# Autodesk Inventor assembly: promo
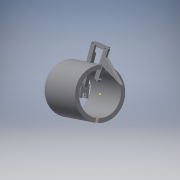
[picture p0: Inventor's stored thumbnail of the model, 180x180]
Saved by Autodesk Inventor 2016 (Build 200138000, 138)
## iProperties
Created: 2016-05-12
Part Number: promo
Material: 一般
Document SubType Name: Assembly
Designer: 宏太
Author: 宏太
## Documents named in this file (6)
- C:\Users\宏太\Documents\Inventor\Content Center Files\Tomoto2016\promo.iam
- C:\Users\宏太\Documents\Inventor\Content Center Files\Tomoto2016\promo_arm2.ipt
- C:\Users\宏太\Documents\Inventor\Content Center Files\Tomoto2016\promo_hold2.ipt
- C:\Users\宏太\Documents\Inventor\Content Center Files\Tomoto2016\promo_arm1.ipt
- C:\Users\宏太\Documents\Inventor\Content Center Files\Tomoto2016\promo_hold.ipt
- C:\Users\宏太\Documents\Inventor\Content Center Files\Tomoto2016\pipe.ipt
## Components (5 placed, 5 different names)
1. promo_arm2:1 — 挿入:2, 挿入:5
2. promo_hold2:1 — 挿入:5
3. promo_arm1:1 — 挿入:2, 挿入:4
4. promo_hold:1 — 挿入:4, 挿入:6
5. pipe:1 — 挿入:6
## Relationships (4: Insert 4)
- 挿入:2 [Insert]: promo_arm2:1 ↔ promo_arm1:1
- 挿入:4 [Insert]: promo_arm1:1 ↔ promo_hold:1
- 挿入:5 [Insert]: promo_arm2:1 ↔ promo_hold2:1
- 挿入:6 [Insert] (30 mm): promo_hold:1 ↔ pipe:1
